# Autodesk Inventor assembly: ASM Main
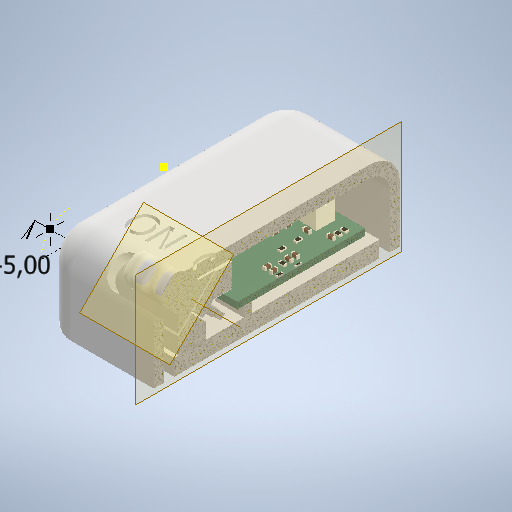
[picture p0: Inventor's stored thumbnail of the model, 512x512]
Saved by Autodesk Inventor 2025.2 (Build 292293000, 293)
## iProperties
Created: 2024-11-12
Part Number: ASM Main
Document SubType Name: Assembly
Designer: matss
Author: matss
## Documents named in this file (6)
- C:\Users\matss\Documents\.Studium\Health_Device\CAD\Wearable-Health-Device\ASM Main.iam
- C:\Users\matss\Documents\.Studium\Health_Device\CAD\Wearable-Health-Device\MCI_PCB\MCI_PCB\MCI_PCB.iam
- C:\Users\matss\Documents\.Studium\Health_Device\CAD\Wearable-Health-Device\PCB_Mount.ipt
- C:\Users\matss\Documents\.Studium\Health_Device\CAD\Wearable-Health-Device\PCB_Deckel.ipt
- C:\Users\matss\Documents\.Studium\Health_Device\CAD\Wearable-Health-Device\Schalter.ipt
- C:\Users\matss\Documents\.Studium\Health_Device\CAD\Wearable-Health-Device\Schalter_vergroeßerung.ipt
## Components (5 placed, 5 different names)
1. MCI_PCB:1 [sub-assembly] — Mate:4, Mate:5, Mate:6
2. PCB_Mount:1 — Mate:1, Mate:2, Mate:3, Mate:4, Mate:5, Mate:6, Mate:7, Mate:8, Flush:10
3. PCB_Deckel:1 — Mate:7, Mate:8, Flush:10, Mate:9, Mate:10
4. Schalter:1 — Mate:12, Mate:15, Mate:16
5. Schalter_vergroeßerung:1 — Mate:9, Mate:10, Mate:12, Mate:15, Mate:16
## Relationships (14: Mate 13, Flush 1)
- Mate:1: PCB_Mount:1
- Mate:2: PCB_Mount:1
- Mate:3 (20 mm): PCB_Mount:1
- Mate:4 (2.5 mm): MCI_PCB:1 ↔ PCB_Mount:1
- Mate:5: MCI_PCB:1 ↔ PCB_Mount:1
- Mate:6: MCI_PCB:1 ↔ PCB_Mount:1
- Mate:7: PCB_Mount:1 ↔ PCB_Deckel:1
- Mate:8: PCB_Mount:1 ↔ PCB_Deckel:1
- Flush:10: PCB_Mount:1 ↔ PCB_Deckel:1
- Mate:9 (0.25 mm): PCB_Deckel:1 ↔ Schalter_vergroeßerung:1
- Mate:10 (0.5 mm): PCB_Deckel:1 ↔ Schalter_vergroeßerung:1
- Mate:12: Schalter:1 ↔ Schalter_vergroeßerung:1
- Mate:15: Schalter:1 ↔ Schalter_vergroeßerung:1
- Mate:16 (0.5 mm): Schalter:1 ↔ Schalter_vergroeßerung:1
